# Autodesk Inventor assembly: astacompleta306
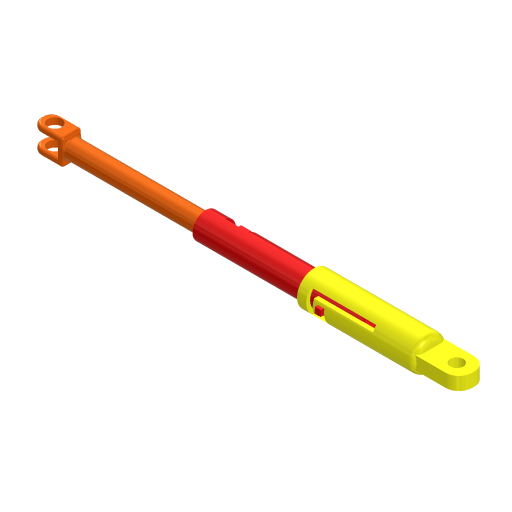
[picture p0: Inventor's stored thumbnail of the model, 512x512]
Saved by Autodesk Inventor 2024 (Build 280153000, 153)
## iProperties
Created: 2024-05-11
Part Number: astacompleta306
Document SubType Name: Assembly
Designer: alexz
Author: alexz
## Documents named in this file (4)
- C:\Users\alexz\Documents\Inventor\Esercizi\Progetto\astacompleta306.iam
- C:\Users\alexz\Documents\Inventor\Esercizi\Progetto\asteoscila1_(306).ipt
- C:\Users\alexz\Documents\Inventor\Esercizi\Progetto\astaoscilla2_306.ipt
- C:\Users\alexz\Documents\Inventor\Esercizi\Progetto\astaoscilla3_(306).ipt
## Components (3 placed, 3 different names)
1. asteoscila1_(306):1 — Cylindrical:1
2. astaoscilla2_306:1 — Cylindrical:1, Cylindrical:2
3. astaoscilla3_(306):1 — Cylindrical:2
## Relationships (2: CylindricalJoint 2)
- Cylindrical:1: asteoscila1_(306):1 ↔ astaoscilla2_306:1
- Cylindrical:2: astaoscilla2_306:1 ↔ astaoscilla3_(306):1
